# Autodesk Inventor assembly: Twitter
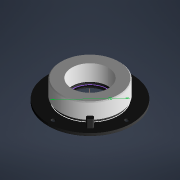
[picture p0: Inventor's stored thumbnail of the model, 180x180]
Saved by Autodesk Inventor 2022 (Build 260153070, 153G)
## iProperties
Created: 2021-11-19
Part Number: Twitter
Document SubType Name: Assembly
Designer: kalugin_a
Author: kalugin_a
## Documents named in this file (4)
- C:\Users\kalugin_a\Documents\Inventor\TUTO\MELAS\Workspace\Twitter.iam
- C:\Users\kalugin_a\Documents\Inventor\TUTO\MELAS\Workspace\Фланец.ipt
- C:\Users\kalugin_a\Documents\Inventor\TUTO\MELAS\Workspace\Clemm.ipt
- C:\Users\kalugin_a\Documents\Inventor\TUTO\MELAS\Workspace\Magnetic.ipt
## Components (6 placed, 3 different names)
1. Фланец:1 — Жесткий:1, Заподлицо:1
2. Magnetic:1 — Заподлицо:1
3. Clemm:1 — Жесткий:1
4. Clemm:2
5. Clemm:3
6. Clemm:4
## Component patterns: (4 elements, first: Clemm:1)
## Relationships (2: WeldJoint 1, Flush 1)
- Жесткий:1 [WeldJoint]: Фланец:1 ↔ Clemm:1
- Заподлицо:1 [Flush]: Фланец:1 ↔ Magnetic:1
